# Autodesk Inventor assembly: camera holder design
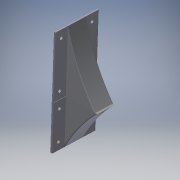
[picture p0: Inventor's stored thumbnail of the model, 180x180]
Saved by Autodesk Inventor 2017 (Build 210142000, 142)
## iProperties
Created: 2016-11-05
Part Number: camera holder design
Document SubType Name: Assembly
Designer: Juan Maldonado
Author: Juan Maldonado
## Documents named in this file (3)
- C:\Users\Juan Maldonado\Documents\TRC\Camera and antenna covers\camera holder design.iam
- C:\Users\Juan Maldonado\Documents\TRC\Camera and antenna covers\top camera cover.ipt
- C:\Users\Juan Maldonado\Documents\TRC\Camera and antenna covers\bottom camera cover.ipt
## Components (2 placed, 2 different names)
1. top camera cover:1 — Mate:1
2. bottom camera cover:1 — Mate:1
## Relationships (1: Mate 1)
- Mate:1: top camera cover:1 ↔ bottom camera cover:1
